# Autodesk Inventor assembly: Rover_2.0
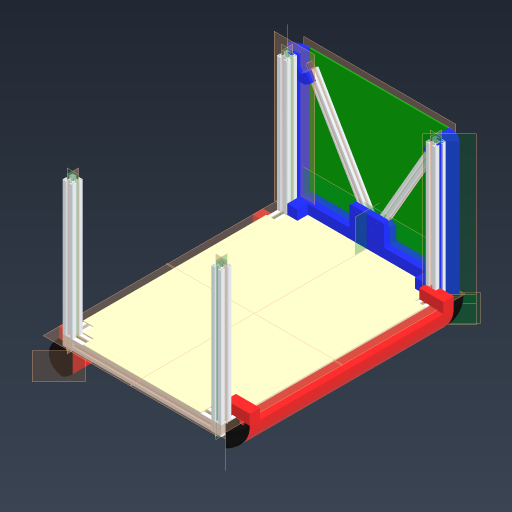
[picture p0: Inventor's stored thumbnail of the model, 512x512]
Saved by Autodesk Inventor 2023.2 (Build 272271030, 271C)
## iProperties
Created: 2025-08-19
Part Number: Rover_2.0
Document SubType Name: Assembly
Designer: Олег Коноваленко
Author: Олег Коноваленко
## Documents named in this file (6)
- D:\!Rover\Rover\Rover_construction\Rover_2.0.iam
- D:\!Rover\Rover\Rover_construction\3-х сторонний соединитель 30х30\3-х сторонний соединитель 30х30.ipt
- D:\!Rover\Rover\Rover_construction\Боковые стены.iam
- D:\!Rover\Rover\Rover_construction\Профиль 30x30\Грубый профиль_30x30.ipt
- D:\!Rover\Rover\Rover_construction\Фанера платформы.ipt
- D:\!Rover\Rover\Rover_construction\Задняя стенка.iam
## Components (16 placed, 5 different names)
1. Боковые стены:2 [sub-assembly] — Совмещение:43
2. Боковые стены:3 [sub-assembly] — Совмещение:44
3. Фанера платформы:1 — Совмещение:46, Заподлицо:22, Заподлицо:23
4. Задняя стенка:1 [sub-assembly] — Совмещение:47, Заподлицо:24, Совмещение:48
5. Грубый профиль_30x30:1 — Заподлицо:1, Совмещение:18, Заподлицо:2, Заподлицо:3, Совмещение:19, Заподлицо:15, Совмещение:44, Совмещение:46, Заподлицо:23
6. Грубый профиль_30x30:2 — Совмещение:30, Совмещение:32, Совмещение:33, Симметрия:1, Симметрия:2, Совмещение:47, Заподлицо:24, Совмещение:48
7. Грубый профиль_30x30:3 — Совмещение:29, Заподлицо:14, Совмещение:37
8. Грубый профиль_30x30:4 — Заподлицо:10, Заподлицо:11, Заподлицо:12, Совмещение:26, Совмещение:27
9. Грубый профиль_30x30:5 — Заподлицо:4, Заподлицо:5, Заподлицо:6, Совмещение:20, Совмещение:21, Совмещение:22, Совмещение:43
10. Грубый профиль_30x30:6 — Совмещение:28, Совмещение:35, Совмещение:36, Симметрия:1, Симметрия:2
11. Грубый профиль_30x30:7 — Совмещение:31, Заподлицо:13, Совмещение:34
12. Грубый профиль_30x30:8 — Совмещение:23, Заподлицо:7, Заподлицо:8, Заподлицо:9, Совмещение:24, Совмещение:25, Заподлицо:22
13. 3-х сторонний соединитель 30х30:2 — Заподлицо:1, Совмещение:18, Заподлицо:2, Заподлицо:10, Заподлицо:11, Совмещение:27, Совмещение:30, Совмещение:32, Совмещение:33
14. 3-х сторонний соединитель 30х30:3 — Заподлицо:6, Совмещение:20, Совмещение:21, Заподлицо:12, Совмещение:26, Совмещение:29, Заподлицо:14, Совмещение:37
15. 3-х сторонний соединитель 30х30:4 — Заподлицо:3, Совмещение:19, Совмещение:23, Заподлицо:7, Совмещение:25, Совмещение:31, Заподлицо:13, Совмещение:34
16. 3-х сторонний соединитель 30х30:1 — Заподлицо:4, Заподлицо:5, Совмещение:22, Заподлицо:8, Заподлицо:9, Совмещение:24, Совмещение:28, Совмещение:35, Совмещение:36
## Relationships (49: Mate 29, Flush 18, Symmetry 2)
- Совмещение:16 [Mate]
- Совмещение:17 [Mate]
- Заподлицо:1 [Flush]: Грубый профиль_30x30:1 ↔ 3-х сторонний соединитель 30х30:2
- Совмещение:18 [Mate]: Грубый профиль_30x30:1 ↔ 3-х сторонний соединитель 30х30:2
- Заподлицо:2 [Flush]: Грубый профиль_30x30:1 ↔ 3-х сторонний соединитель 30х30:2
- Заподлицо:3 [Flush]: Грубый профиль_30x30:1 ↔ 3-х сторонний соединитель 30х30:4
- Совмещение:19 [Mate]: Грубый профиль_30x30:1 ↔ 3-х сторонний соединитель 30х30:4
- Заподлицо:4 [Flush]: Грубый профиль_30x30:5 ↔ 3-х сторонний соединитель 30х30:1
- Заподлицо:5 [Flush]: Грубый профиль_30x30:5 ↔ 3-х сторонний соединитель 30х30:1
- Заподлицо:6 [Flush]: Грубый профиль_30x30:5 ↔ 3-х сторонний соединитель 30х30:3
- Совмещение:20 [Mate]: Грубый профиль_30x30:5 ↔ 3-х сторонний соединитель 30х30:3
- Совмещение:21 [Mate]: Грубый профиль_30x30:5 ↔ 3-х сторонний соединитель 30х30:3
- Совмещение:22 [Mate]: Грубый профиль_30x30:5 ↔ 3-х сторонний соединитель 30х30:1
- Совмещение:23 [Mate]: Грубый профиль_30x30:8 ↔ 3-х сторонний соединитель 30х30:4
- Заподлицо:7 [Flush]: Грубый профиль_30x30:8 ↔ 3-х сторонний соединитель 30х30:4
- Заподлицо:8 [Flush]: Грубый профиль_30x30:8 ↔ 3-х сторонний соединитель 30х30:1
- Заподлицо:9 [Flush]: Грубый профиль_30x30:8 ↔ 3-х сторонний соединитель 30х30:1
- Совмещение:24 [Mate]: Грубый профиль_30x30:8 ↔ 3-х сторонний соединитель 30х30:1
- Совмещение:25 [Mate]: Грубый профиль_30x30:8 ↔ 3-х сторонний соединитель 30х30:4
- Заподлицо:10 [Flush]: Грубый профиль_30x30:4 ↔ 3-х сторонний соединитель 30х30:2
- Заподлицо:11 [Flush]: Грубый профиль_30x30:4 ↔ 3-х сторонний соединитель 30х30:2
- Заподлицо:12 [Flush]: Грубый профиль_30x30:4 ↔ 3-х сторонний соединитель 30х30:3
- Совмещение:26 [Mate]: Грубый профиль_30x30:4 ↔ 3-х сторонний соединитель 30х30:3
- Совмещение:27 [Mate]: Грубый профиль_30x30:4 ↔ 3-х сторонний соединитель 30х30:2
- Совмещение:28 [Mate]: Грубый профиль_30x30:6 ↔ 3-х сторонний соединитель 30х30:1
- Совмещение:29 [Mate]: Грубый профиль_30x30:3 ↔ 3-х сторонний соединитель 30х30:3
- Совмещение:30 [Mate]: Грубый профиль_30x30:2 ↔ 3-х сторонний соединитель 30х30:2
- Совмещение:31 [Mate]: Грубый профиль_30x30:7 ↔ 3-х сторонний соединитель 30х30:4
- Совмещение:32 [Mate]: Грубый профиль_30x30:2 ↔ 3-х сторонний соединитель 30х30:2
- Совмещение:33 [Mate]: Грубый профиль_30x30:2 ↔ 3-х сторонний соединитель 30х30:2
- Заподлицо:13 [Flush]: Грубый профиль_30x30:7 ↔ 3-х сторонний соединитель 30х30:4
- Совмещение:34 [Mate]: Грубый профиль_30x30:7 ↔ 3-х сторонний соединитель 30х30:4
- Совмещение:35 [Mate]: Грубый профиль_30x30:6 ↔ 3-х сторонний соединитель 30х30:1
- Совмещение:36 [Mate]: Грубый профиль_30x30:6 ↔ 3-х сторонний соединитель 30х30:1
- Заподлицо:14 [Flush]: Грубый профиль_30x30:3 ↔ 3-х сторонний соединитель 30х30:3
- Совмещение:37 [Mate]: Грубый профиль_30x30:3 ↔ 3-х сторонний соединитель 30х30:3
- Заподлицо:15 [Flush]: Грубый профиль_30x30:1
- Симметрия:1 [Symmetry]: Грубый профиль_30x30:2 ↔ Грубый профиль_30x30:6
- Совмещение:38 [Mate]
- Симметрия:2 [Symmetry]: Грубый профиль_30x30:2 ↔ Грубый профиль_30x30:6
- Совмещение:39 [Mate]
- Совмещение:43 [Mate]: Боковые стены:2 ↔ Грубый профиль_30x30:5
- Совмещение:44 [Mate]: Боковые стены:3 ↔ Грубый профиль_30x30:1
- Совмещение:46 [Mate]: Фанера платформы:1 ↔ Грубый профиль_30x30:1
- Заподлицо:22 [Flush]: Фанера платформы:1 ↔ Грубый профиль_30x30:8
- Заподлицо:23 [Flush]: Фанера платформы:1 ↔ Грубый профиль_30x30:1
- Совмещение:47 [Mate]: Задняя стенка:1 ↔ Грубый профиль_30x30:2
- Заподлицо:24 [Flush]: Задняя стенка:1 ↔ Грубый профиль_30x30:2
- Совмещение:48 [Mate]: Задняя стенка:1 ↔ Грубый профиль_30x30:2
